# Autodesk Inventor assembly: Shaft Collar Set Screw_MIR6
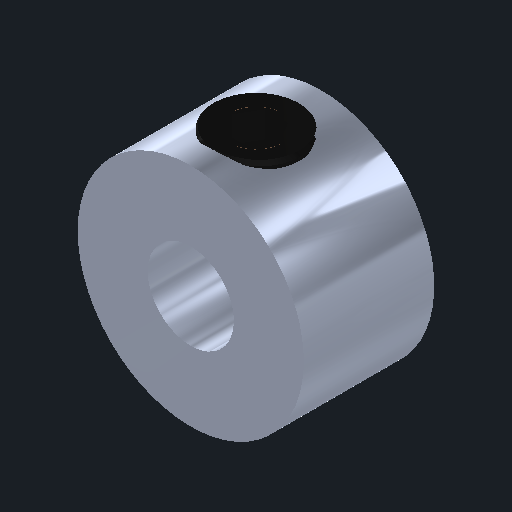
[picture p0: Inventor's stored thumbnail of the model, 512x512]
Saved by Autodesk Inventor 2024 (Build 280153000, 153)
## iProperties
Created: 2022-08-01
Part Number: Shaft Collar Set Screw_MIR6
Document SubType Name: Assembly
Designer: macbook
Author: ylu12
## Documents named in this file (3)
- \\Mac\Home\Desktop\code\1599V-VRC\Cad\Motion\Shaft LS\Shaft Collar Metal\Shaft Collar Set Screw_MIR6.iam
- \\Mac\Home\Desktop\code\1599V-VRC\Cad\Motion\Reference Files\Shaft Collar Metal_MIR7.ipt
- \\Mac\Home\Desktop\code\1599V-VRC\Cad\Motion\Reference Files\Set Screw_MIR6.ipt
## Components (2 placed, 2 different names)
1. Shaft Collar Metal_MIR7:1 — Flush:1, Mate:2, Mate:1, Insert:1
2. Set Screw_MIR6:1 — Insert:1
## Relationships (4: Mate 2, Flush 1, Insert 1)
- Flush:1: Shaft Collar Metal_MIR7:1
- Mate:2: Shaft Collar Metal_MIR7:1
- Mate:1: Shaft Collar Metal_MIR7:1
- Insert:1: Shaft Collar Metal_MIR7:1 ↔ Set Screw_MIR6:1
